# Autodesk Inventor assembly: Sfu1000
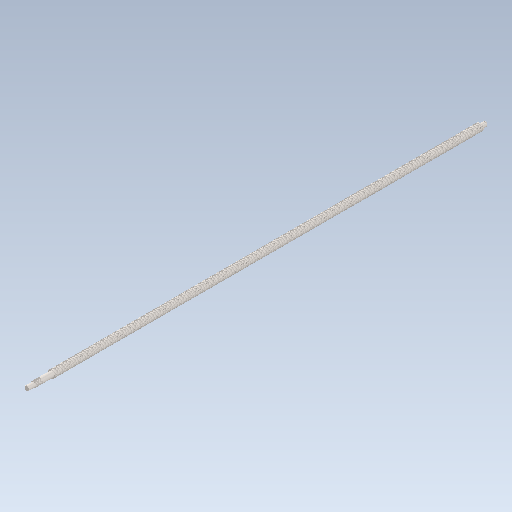
[picture p0: Inventor's stored thumbnail of the model, 512x512]
Saved by Autodesk Inventor 2020.1 (Build 241239000, 239)
## iProperties
Created: 2023-01-06
Part Number: Sfu1000
Document SubType Name: Assembly
Designer: KirikDK
Mass: 50.1165 g
Surface Area: 186.532 cm^2
Volume: 50.1165 cm^3
Density: 1 g/cm^3
Author: KirikDK
## Documents named in this file (3)
- C:\Users\KirikDK\Documents\Stanik1000\Sfu1000.iam
- C:\Users\KirikDK\Documents\Stanik1000\SfuObrezki\SFU1605-300end.ipt
- C:\Users\KirikDK\Documents\Stanik1000\SfuObrezki\SFU1605-700start.ipt
## Components (2 placed, 2 different names)
1. SFU1605-300end:1 — Совмещение:1, Совмещение:2
2. SFU1605-700start:1 — Совмещение:1, Совмещение:2
## Relationships (2: Mate 2)
- Совмещение:1 [Mate]: SFU1605-300end:1 ↔ SFU1605-700start:1
- Совмещение:2 [Mate]: SFU1605-300end:1 ↔ SFU1605-700start:1
